# Autodesk Inventor assembly: Aero_assembly
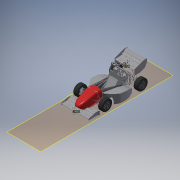
[picture p0: Inventor's stored thumbnail of the model, 180x180]
Saved by Autodesk Inventor 2018.3 (Build 223284000, 284)
## iProperties
Created: 2018-03-12
Part Number: Aero_assembly
Material: 一般
Document SubType Name: Assembly
Designer: ku_sk
Author: ku_sk
## Documents named in this file (20)
- D:\ku_sk\ドキュメント\Inventor\Aero\KS-15\Aero_assembly.iam
- D:\ku_sk\ドキュメント\Inventor\Aero\KS-15\Fr.wing\Fr.wing_assy.iam
- D:\ku_sk\ドキュメント\Inventor\Aero\KS-15\Rr.wing\Rr.wing_assy.iam
- D:\ku_sk\ドキュメント\Inventor\Aero\KS-15\body\2018 zentai assembly.iam
- D:\ku_sk\ドキュメント\Inventor\Aero\KS-15\Pontoon\2018 radiator analysis.iam
- D:\ku_sk\ドキュメント\Inventor\Aero\KS-15\body\parts\2015Wheel watanabe.ipt
- D:\ku_sk\ドキュメント\Inventor\Aero\KS-15\Rr.wing\parts\stay\collar_6.2.ipt
- D:\ku_sk\ドキュメント\Inventor\Aero\KS-15\Rr.wing\parts\stay\end\parts\Symmetry of POS_8ECBall.ipt
- D:\ku_sk\ドキュメント\Inventor\Aero\KS-15\Rr.wing\parts\stay\end\stay end.iam
- D:\ku_sk\ドキュメント\Inventor\Aero\KS-15\Rr.wing\parts\stay\stay1.iam
- D:\ku_sk\ドキュメント\Inventor\Aero\KS-15\Rr.wing\parts\stay\stay2.iam
- D:\ku_sk\ドキュメント\Inventor\Aero\KS-15\Rr.wing\parts\stay\stay3.iam
- D:\ku_sk\ドキュメント\Inventor\Aero\KS-15\Rr.wing\parts\stay\collar_4.2.ipt
- D:\ku_sk\ドキュメント\Inventor\Aero\KS-15\Rr.wing\parts\stay\collar_6.21.ipt
- D:\ku_sk\ドキュメント\Inventor\Aero\KS-15\Rr.wing\parts\stay\end\parts\Symmetry of POS_8ECBall2.ipt
- D:\ku_sk\ドキュメント\Inventor\Aero\KS-15\Rr.wing\parts\stay\end\stay end2.iam
- D:\ku_sk\ドキュメント\Inventor\Aero\KS-15\Rr.wing\parts\stay\stay12.iam
- D:\ku_sk\ドキュメント\Inventor\Aero\KS-15\Rr.wing\parts\stay\stay22.iam
- D:\ku_sk\ドキュメント\Inventor\Aero\KS-15\Rr.wing\parts\stay\stay32.iam
- D:\ku_sk\ドキュメント\Inventor\Aero\KS-15\Rr.wing\parts\stay\collar_4.21.ipt
## Components (36 placed, 19 different names)
1. 2018 zentai assembly:1 [sub-assembly] — メイト:8, メイト:9, メイト:10, メイト:14, メイト:15, フラッシュ:9, フラッシュ:10, メイト:18, メイト:19, メイト:20, メイト:21, メイト:22, メイト:23, メイト:30, メイト:31, メイト:32, メイト:33
2. 2018 radiator analysis:1 [sub-assembly] — メイト:11, メイト:12, メイト:13
3. Fr.wing_assy:1 [sub-assembly] — フラッシュ:1
4. Rr.wing_assy:1 [sub-assembly] — フラッシュ:6, ボール:1, ボール:6, ボール:7
5. 2015Wheel watanabe:1 — メイト:14, フラッシュ:10
6. 2015Wheel watanabe:2 — メイト:15, フラッシュ:9
7. collar_6.2:1 — メイト:16, メイト:19, メイト:20, メイト:24, メイト:26
8. collar_6.2:2 — メイト:17, メイト:18, メイト:21, メイト:25, メイト:27
9. collar_6.2:3 — メイト:16, メイト:23
10. collar_6.2:4 — メイト:17, メイト:22
11. Symmetry of POS_8ECBall:1 — メイト:25, メイト:27, ボール:4
12. Symmetry of POS_8ECBall:2 — メイト:24, メイト:26, ボール:5
13. stay end:1 [sub-assembly] — ボール:4, メイト:28
14. stay end:2 [sub-assembly] — ボール:5, メイト:29
15. stay end:3 [sub-assembly] — ボール:8, メイト:36
16. stay1:1 [sub-assembly] — ボール:6, メイト:28
17. stay2:1 [sub-assembly] — ボール:7, メイト:29
18. stay3:1 [sub-assembly] — ボール:1, メイト:36
19. collar_4.2:1 — メイト:32, メイト:33, メイト:35
20. collar_4.2:2 — メイト:30, メイト:31, メイト:34
21. Symmetry of POS_8ECBall:3 — メイト:34, メイト:35, ボール:8
22. collar_6.21:1 — メイト:37, メイト:41, メイト:42
23. collar_6.21:2 — メイト:38, メイト:39, メイト:40
24. collar_6.21:3 — メイト:37
25. collar_6.21:4 — メイト:38
26. Symmetry of POS_8ECBall2:1 — メイト:39, メイト:40, ボール:9
27. Symmetry of POS_8ECBall2:2 — メイト:41, メイト:42, ボール:10
28. stay end2:1 [sub-assembly] — メイト:43, ボール:9
29. stay end2:2 [sub-assembly] — メイト:44, ボール:10
30. stay end2:3 [sub-assembly] — メイト:45, ボール:11
31. stay12:1 [sub-assembly] — メイト:43
32. stay22:1 [sub-assembly] — メイト:44
33. stay32:1 [sub-assembly] — メイト:45
34. collar_4.21:1 — メイト:46
35. collar_4.21:2 — メイト:47
36. Symmetry of POS_8ECBall2:3 — メイト:46, メイト:47, ボール:11
## Relationships (54: Mate 40, BallJoint 9, Flush 5)
- フラッシュ:1 [Flush]: Fr.wing_assy:1
- フラッシュ:6 [Flush]: Rr.wing_assy:1
- メイト:8 [Mate]: 2018 zentai assembly:1
- メイト:9 [Mate]: 2018 zentai assembly:1
- メイト:10 [Mate]: 2018 zentai assembly:1
- メイト:11 [Mate]: 2018 radiator analysis:1
- メイト:12 [Mate]: 2018 radiator analysis:1
- メイト:13 [Mate]: 2018 radiator analysis:1
- メイト:14 [Mate]: 2018 zentai assembly:1 ↔ 2015Wheel watanabe:1
- メイト:15 [Mate]: 2018 zentai assembly:1 ↔ 2015Wheel watanabe:2
- フラッシュ:9 [Flush]: 2018 zentai assembly:1 ↔ 2015Wheel watanabe:2
- フラッシュ:10 [Flush]: 2018 zentai assembly:1 ↔ 2015Wheel watanabe:1
- フラッシュ:11 [Flush] (22.861 mm)
- メイト:16 [Mate]: collar_6.2:1 ↔ collar_6.2:3
- メイト:17 [Mate]: collar_6.2:2 ↔ collar_6.2:4
- メイト:18 [Mate]: 2018 zentai assembly:1 ↔ collar_6.2:2
- メイト:19 [Mate]: 2018 zentai assembly:1 ↔ collar_6.2:1
- メイト:20 [Mate]: 2018 zentai assembly:1 ↔ collar_6.2:1
- メイト:21 [Mate]: 2018 zentai assembly:1 ↔ collar_6.2:2
- メイト:22 [Mate]: 2018 zentai assembly:1 ↔ collar_6.2:4
- メイト:23 [Mate]: 2018 zentai assembly:1 ↔ collar_6.2:3
- メイト:24 [Mate]: collar_6.2:1 ↔ Symmetry of POS_8ECBall:2
- メイト:25 [Mate]: collar_6.2:2 ↔ Symmetry of POS_8ECBall:1
- メイト:26 [Mate]: collar_6.2:1 ↔ Symmetry of POS_8ECBall:2
- メイト:27 [Mate]: collar_6.2:2 ↔ Symmetry of POS_8ECBall:1
- ボール:1 [BallJoint]: Rr.wing_assy:1 ↔ stay3:1
- ボール:4 [BallJoint]: Symmetry of POS_8ECBall:1 ↔ stay end:1
- ボール:5 [BallJoint]: Symmetry of POS_8ECBall:2 ↔ stay end:2
- ボール:6 [BallJoint]: Rr.wing_assy:1 ↔ stay1:1
- ボール:7 [BallJoint]: Rr.wing_assy:1 ↔ stay2:1
- メイト:28 [Mate]: stay end:1 ↔ stay1:1
- メイト:29 [Mate]: stay end:2 ↔ stay2:1
- メイト:30 [Mate]: 2018 zentai assembly:1 ↔ collar_4.2:2
- メイト:31 [Mate]: 2018 zentai assembly:1 ↔ collar_4.2:2
- メイト:32 [Mate]: 2018 zentai assembly:1 ↔ collar_4.2:1
- メイト:33 [Mate]: 2018 zentai assembly:1 ↔ collar_4.2:1
- メイト:34 [Mate]: collar_4.2:2 ↔ Symmetry of POS_8ECBall:3
- メイト:35 [Mate]: collar_4.2:1 ↔ Symmetry of POS_8ECBall:3
- ボール:8 [BallJoint]: stay end:3 ↔ Symmetry of POS_8ECBall:3
- メイト:36 [Mate]: stay end:3 ↔ stay3:1
- メイト:37 [Mate]: collar_6.21:1 ↔ collar_6.21:3
- メイト:38 [Mate]: collar_6.21:2 ↔ collar_6.21:4
- メイト:39 [Mate]: collar_6.21:2 ↔ Symmetry of POS_8ECBall2:1
- メイト:40 [Mate]: collar_6.21:2 ↔ Symmetry of POS_8ECBall2:1
- メイト:41 [Mate]: collar_6.21:1 ↔ Symmetry of POS_8ECBall2:2
- メイト:42 [Mate]: collar_6.21:1 ↔ Symmetry of POS_8ECBall2:2
- メイト:43 [Mate]: stay end2:1 ↔ stay12:1
- メイト:44 [Mate]: stay end2:2 ↔ stay22:1
- メイト:45 [Mate]: stay end2:3 ↔ stay32:1
- メイト:46 [Mate]: collar_4.21:1 ↔ Symmetry of POS_8ECBall2:3
- メイト:47 [Mate]: collar_4.21:2 ↔ Symmetry of POS_8ECBall2:3
- ボール:9 [BallJoint]: Symmetry of POS_8ECBall2:1 ↔ stay end2:1
- ボール:10 [BallJoint]: Symmetry of POS_8ECBall2:2 ↔ stay end2:2
- ボール:11 [BallJoint]: stay end2:3 ↔ Symmetry of POS_8ECBall2:3
